# Autodesk Inventor assembly: ImagineFrameV2
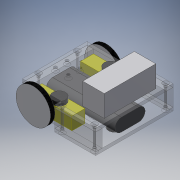
[picture p0: Inventor's stored thumbnail of the model, 180x180]
Saved by Autodesk Inventor 2018 (Build 220112000, 112)
## iProperties
Created: 2020-09-26
Part Number: ImagineFrameV2
Document SubType Name: Assembly
Designer: Lveli
Author: Lveli
## Documents named in this file (9)
- C:\Users\Lveli\Documents\CAD\ritimagine\FrameV2\ImagineFrameV2.iam
- C:\Users\Lveli\Documents\CAD\ritimagine\FrameV2\ImagineFrameTopBot.ipt
- C:\Users\Lveli\Documents\CAD\ritimagine\FrameV2\ImagineFrameSides.ipt
- C:\Users\Lveli\Documents\CAD\ritimagine\FrameV2\ImagineFrameFront.ipt
- C:\Users\Lveli\Documents\CAD\ritimagine\FrameV2\mockmotor.ipt
- C:\Users\Lveli\Documents\CAD\ritimagine\FrameV2\mockbattery.ipt
- C:\Users\Lveli\Documents\CAD\ritimagine\FrameV2\mockPi.ipt
- C:\Users\Lveli\Documents\CAD\ritimagine\FrameV2\FeltPad.ipt
- C:\Users\Lveli\Documents\CAD\ritimagine\FrameV2\mockWheel.ipt
## Components (14 placed, 8 different names)
1. ImagineFrameTopBot:1 — Mate:1, Mate:2, Mate:3, Mate:4, Mate:5, Mate:6, Mate:13, Mate:14, Mate:25, Flush:3, Mate:27, Mate:28, Mate:29, Mate:30
2. ImagineFrameSides:1 — Mate:4, Mate:5, Mate:6, Mate:7, Mate:12
3. ImagineFrameSides:2 — Mate:1, Mate:2, Mate:3, Mate:11
4. ImagineFrameTopBot:2 — Mate:7, Mate:10, Mate:11, Mate:12, Flush:1, Mate:19, Flush:2, Mate:20, Mate:22, Mate:31, Tangent:3
5. ImagineFrameFront:1 — Mate:10, Mate:13, Mate:14, Mate:18, Mate:21, Mate:23, Mate:24, Tangent:1, Tangent:2, Mate:35
6. FeltPad:1 — Mate:27, Mate:30, Tangent:2
7. FeltPad:2 — Mate:28, Mate:29, Tangent:1
8. FeltPad:3 — Mate:31, Mate:32, Tangent:3
9. mockWheel:1 — Mate:33, Mate:34, Mate:35, Mate:36
10. mockWheel:2 — Mate:36, Mate:37
11. mockmotor:1 — Mate:18, Flush:1, Mate:19, Mate:33, Mate:34
12. mockmotor:2 — Flush:2, Mate:20, Mate:21, Mate:37
13. mockbattery:1 — Mate:22, Mate:23, Mate:24, Mate:26, Mate:32
14. mockPi:1 — Mate:25, Mate:26, Flush:3
## Relationships (38: Mate 32, Flush 3, Tangent 3)
- Mate:1: ImagineFrameTopBot:1 ↔ ImagineFrameSides:2
- Mate:2: ImagineFrameTopBot:1 ↔ ImagineFrameSides:2
- Mate:3: ImagineFrameTopBot:1 ↔ ImagineFrameSides:2
- Mate:4: ImagineFrameTopBot:1 ↔ ImagineFrameSides:1
- Mate:5: ImagineFrameTopBot:1 ↔ ImagineFrameSides:1
- Mate:6: ImagineFrameTopBot:1 ↔ ImagineFrameSides:1
- Mate:7: ImagineFrameSides:1 ↔ ImagineFrameTopBot:2
- Mate:10: ImagineFrameTopBot:2 ↔ ImagineFrameFront:1
- Mate:11: ImagineFrameSides:2 ↔ ImagineFrameTopBot:2
- Mate:12: ImagineFrameSides:1 ↔ ImagineFrameTopBot:2
- Mate:13: ImagineFrameTopBot:1 ↔ ImagineFrameFront:1
- Mate:14: ImagineFrameTopBot:1 ↔ ImagineFrameFront:1
- Mate:18: ImagineFrameFront:1 ↔ mockmotor:1
- Flush:1: ImagineFrameTopBot:2 ↔ mockmotor:1
- Mate:19: ImagineFrameTopBot:2 ↔ mockmotor:1
- Flush:2: ImagineFrameTopBot:2 ↔ mockmotor:2
- Mate:20: ImagineFrameTopBot:2 ↔ mockmotor:2
- Mate:21: ImagineFrameFront:1 ↔ mockmotor:2
- Mate:22: ImagineFrameTopBot:2 ↔ mockbattery:1
- Mate:23: ImagineFrameFront:1 ↔ mockbattery:1
- Mate:24 (-47.625 mm): ImagineFrameFront:1 ↔ mockbattery:1
- Mate:25: ImagineFrameTopBot:1 ↔ mockPi:1
- Mate:26: mockbattery:1 ↔ mockPi:1
- Flush:3 (6.35 mm): ImagineFrameTopBot:1 ↔ mockPi:1
- Mate:27: ImagineFrameTopBot:1 ↔ FeltPad:1
- Mate:28: ImagineFrameTopBot:1 ↔ FeltPad:2
- Mate:29 (-9.525 mm): ImagineFrameTopBot:1 ↔ FeltPad:2
- Mate:30 (-9.525 mm): ImagineFrameTopBot:1 ↔ FeltPad:1
- Tangent:1 (25.4 mm): ImagineFrameFront:1 ↔ FeltPad:2
- Tangent:2 (25.4 mm): ImagineFrameFront:1 ↔ FeltPad:1
- Mate:31: ImagineFrameTopBot:2 ↔ FeltPad:3
- Mate:32: FeltPad:3 ↔ mockbattery:1
- Tangent:3 (-38.1 mm): ImagineFrameTopBot:2 ↔ FeltPad:3
- Mate:33 (-9.525 mm): mockWheel:1 ↔ mockmotor:1
- Mate:34: mockWheel:1 ↔ mockmotor:1
- Mate:35 (12.7 mm): ImagineFrameFront:1 ↔ mockWheel:1
- Mate:36: mockWheel:1 ↔ mockWheel:2
- Mate:37: mockWheel:2 ↔ mockmotor:2
